# Autodesk Inventor assembly: 0070.011
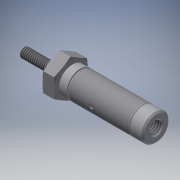
[picture p0: Inventor's stored thumbnail of the model, 180x180]
Saved by Autodesk Inventor 2018 (Build 220112000, 112)
## iProperties
Category: PARTsolutions
Company: BIMBA
Created: 2019-01-16
Part Number: 0070.011
Catalog Web Link: www.cadenas.de
Description: Original Line Standard Air Cylinders-Standard Air Cylinders
Vendor: BIMBA
Document SubType Name: Assembly
Designer: s-4008082
Manufacturer: BIMBA
Mass: 2.26488 g
Surface Area: 33.2461 cm^2
Volume: 2.26488 cm^3
Density: 1 g/cm^3
Title: 0070.011
Author: Cadenas PARTsolutions
Comments: Standard Air Cylinders
PSOL_IDENT_0: {$CADENAS_DATA\23d-libs\bimba\bimba\bimba_imperial\bimba_full_line\original_line_cylinders\standard_
PSOL_IDENT_1: air_cylinders\standard_air_cylinder_asmtab.prj},324 {VTYP=3D},{STYP=ASSTAB},{NB=0070.011},{LINA=0070
PSOL_IDENT_2: .011},{NN=Original Line Standard Air Cylinders},{DATE=21.03.2018 14:31:21},{GEOMDATE=19.03.2018 11:3
PSOL_IDENT_3: 9:15},{VERSION=},{LINEID=20},{WBVAR=STROKE,ACTING,MNT,DER,NR,BM,CO,OO,VO,M,EE,EEL,K,Q,Y,G,T,HL,B,H,S
PSOL_IDENT_4: ER,SR,NT,W,STPT1,STPT2,STPT3,STPT4,MB,PB,PRC,TB,MN},{WBNUMERIC=STROKE,EEL}  {NB=0070.011},{LINA=0070
PSOL_IDENT_5: .011},{KT=DUMMY},{PN=0070.011},{PNC=0070.011},{PNA=(NO ACCESSORIES)},{DASH=},{BORE1=0.31250000},{BOR
PSOL_IDENT_6: E=5/16\" (007)},{BOREPN=007},{STROKE=0.011},{STROKEALG=[0.011:50/0.001]},{STROKE1=0.011},{ACTING=},{
PSOL_IDENT_7: ACTINGALG= '' , 'Single Acting (SA)' , 'R' , 'Reverse Single Acting (SA)' , 'D' , 'Double Acting (SA
PSOL_IDENT_8: )' },{ACTINGPN=},{MNT=},{MNTALG= '' , 'Front Nose Mounting (SA)' , 'XP' , 'Double End or Rear Pivot
PSOL_IDENT_9: Mounting (SA)' },{TYPE=},{MNTPN=},{DER=},{DERALG= '' , 'N/A' },{NR=},{NRALG= '' , 'N/A' },{NRPN=},{B
PSOL_IDENT_10: M=},{BMALG= '' , 'N/A' },{BMPN=},{CO=},{COALG= '' , 'N/A' },{OO=},{OOALG= '', 'N/A' },{OOPN=},{VO=Z}
PSOL_IDENT_11: ,{VOALG= 'Z' , 'N/A' },{VOPN=},{OOVOPN=},{M=},{MALG= '', 'Without Magnet', 'M', 'With Magnet' },{EE=
PSOL_IDENT_12: },{EEL=0.000},{EEMAX=49.9890},{EEALG= '', 'Without Extra Extension', 'EE', 'With Extra Extension' },
PSOL_IDENT_13: {EELALG=0},{EEPN=},{EEPN1=0.000},{K=},{KALG= '' , 'N/A' },{KPN=},{Q=},{QALG= '' , 'Standard Port' , '
PSOL_IDENT_14: Q' , 'Side Port' },{QPN=},{Y=},{YALG= '' , 'N/A' },{YPN=},{YCON=},{F=},{FALG= '', 'Non-Coated (Stand
PSOL_IDENT_15: ard)', 'F', 'Molycoated' },{FPN=},{G=},{GPN=},{GPN99=},{T=},{TALG= '' , 'Standard -20° to 200°F (-29
PSOL_IDENT_16: ° to 95°C)' , 'N' , 'Low Temperature' , 'V' , 'High Temperature' },{NPN=},{VPN=},{HL=},{HLALG= '' , '
PSOL_IDENT_17: N/A' },{B=},{BALG= '' , 'Standard Bumpers' },{BPN=},{H=},{HALG= '', 'N/A' },{HPN=},{SER=},{SERALG= ''
PSOL_IDENT_18: , 'N/A' },{SR=},{SRALG= '' , 'Standard Stainless Steel' },{SRPN=},{SRCON=0},{NT=},{NTPN=},{W=},{WAL
PSOL_IDENT_19: G= '' , 'N/A' },{WPN=},{E=},{EALG= '' , 'Standard Seals/Lube' , 'E' , 'Non-Lube Seals/Lube' },{EPN=}
PSOL_IDENT_20: ,{ST=},{STALG= '' , 'N/A' },{STPT1=},{STPT1ALG= '' , 'N/A' },{STPT2=},{STPT2ALG= '' , 'N/A' },{STPT3=
PSOL_IDENT_21: },{STPT3ALG= '' , 'N/A' },{STPT4=},{STPT4ALG= '' , 'N/A' },{STPN=},{MB=},{MBALG= '' , 'Without Mount
PSOL_IDENT_22: ing Bracket' , 'F,D-26731' , 'D-26731 (front)' },{MBPN=},{MBPNALL=D-26731},{MBPNALLREAR=},{PB=},{PBA
PSOL_IDENT_23: LG= '' , 'N/A' },{PBPN=},{PBPNALL=},{PRC=},{PRCALG= '' , 'W/out Pivot Rod Clevis' , 'F,D-26690' , 'D
PSOL_IDENT_24: -26690 (front)' },{PRCPN=},{PRCPNALL=D-26690},{TB=},{TBALG= '' , 'N/A' },{TBPN=},{TBPNALL=},{MN=},{M
PSOL_IDENT_25: NALG= '' , 'N/A' },{MNPN=},{MNCONF=},{MNCONR=},{TLEN=0.7975},{FRAC=1.3810},{RGCON=},{RGDACCON=},{RHC
PSOL_IDENT_26: ON=},{RHCON1=},{RHCONON=1},{RHACCON=},{FNUTCON=1},{RNUTCON=0},{FNUTPN=D-344},{RNUTPN=},{FNUTTRANS=0.
PSOL_IDENT_27: 0000},{RNUTTRANS=0.0000},{VHOLECON=2},{A1=0.6250},{A1N=0.6250},{A1P=0.8450},{A1B=0.9060},{A4=0.2550}
PSOL_IDENT_28: ,{A4N=0.2550},{A4P=0.1585},{A5=0.0220},{A1H=0.328},{A1NH=0.3280},{A1PH=0.8750},{A1BH=0.0000},{A1SH=0
PSOL_IDENT_29: .0000},{A2H=0.1585},{A2NH=0.1585},{LENGTH=1.1200},{LENGTH1=1.1200},{LENGTH2=1.6500},{MUL=0.0083},{MU
PSOL_IDENT_30: L11=0.0083},{MUL22=0.01375},{MUL33=0.0083},{MUL2=0.7500},{MUL211=0.7500},{MUL222=1.2500},{MUL233=0.7
PSOL_IDENT_31: 500},{SSS=0.0110},{RGLEN=0.3920},{RHLEN=0.1915},{SSS1=1.0000},{A13=0.7190},{DIF=0.0000},{G5=0.0000},
PSOL_IDENT_32: {ON=0},{SSADD=0.0000},{BADD=0.0000},{MADD=0.0000},{NVADD=0.0000},{TRACKL=0.4915},{TRACKCON=D-74168},
PSOL_IDENT_33: {TRIMCON=0},{TRIMCON1=0},{PINCON=},{FSPACE=0.2998},{SPACE=0.0179},{TEXT=0.0313},{S1=0.5000},{D1=0.35
PSOL_IDENT_34: 90},{D1N=0.3590},{D1B=0.6050},{D1P=0.0000},{FA=0.440},{RA=0.0000},{PPATH=standard_air_cylinder_asmtp
PSOL_IDENT_35: l.prj},{MATALGHTML=<b>Standard Original Line:</b><dl><dt>Rod:</dt><dd>- Stainless Steel</dd><dd>&nbs
PSOL_IDENT_36: p;&nbsp;(5/16 9/16 Bores)</dd><dd>- High Strength Carbon Steel</dd><dd>&nbsp;&nbsp;(3/4 3 Bore)</dd>
PSOL_IDENT_37: <dd>- Stainless Steel</dd><dd>&nbsp;&nbsp;(X style DXP/DX/DXDE)</dd><dt>Bearings:</dt><dd>- Sintered
PSOL_IDENT_38: Bronze</dd><dt>Body:</dt><dd>- 304 Stainless Steel</dd><dt>End Caps:</dt><dd>- Aluminum</dd><dt>Sea
PSOL_IDENT_39: ls:</dt><dd>- Buna N</dd></dl>},{ASSCFGPRA=007},{MBPNA=},{MNPNA=},{PRCPNA=},{ASSOPTACC=STPT4},{A=1.3
PSOL_IDENT_40: 8},{HADD=0.0000},{WFL=0},{QADD=0.000},{QADD1=0.200},{TEST=0.0000},{MNTB=},{STDNUTF=1},{STDNUTR=0},{S
PSOL_IDENT_41: TRK2D=0},{X2D=2},{STROKESW=0.011},{EESW=0.000},{FCD=0},{BCD=0},{RCD=0},{CUSTADD=0.000},{FT=#5-40},{F
PSOL_IDENT_42: T1=#5-40},{FT2=3/8-24 UNF-2A},{PORT=#10-32},{FT11=1/2-28 UNF-2A},{FT12=3/8-24 UNF-2A},{B1=}
NN: Original Line Standard Air Cylinders
NT: Standard Male Thread
NB: 0070.011
NBSYN: $PNC.
LINA: 0070.011
PN: 0070.011
PNA: (NO ACCESSORIES)
BORE: 5/16" (007)
STROKE: 0.011
ACTING: Standard Single
MNT: Standard Front Nose
DER: N/A
NR: N/A
BM: N/A
CO: N/A
OO: N/A
VO: N/A
M: Without Magnet Piston
EE: Standard Rod Extension
EEL: 0
K: N/A
Q: Standard Axial Port
Y: N/A
G: Standard Grease Lube
T: Standard -20° to 200°F (-29° to 95°C)
HL: N/A
B: Standard Bumpers
H: N/A
SER: N/A
SR: Standard Stainless Steel
W: N/A
STPT1: N/A
STPT2: N/A
STPT3: N/A
STPT4: N/A
MB: Without Mounting Bracket
PB: N/A
PRC: Without Piston Rod Clevis
TB: N/A
MN: N/A
A: 1.38
SUPPLIER: BIMBA
ARTICLENO: 0070.011
BOMINFO: 0070.011
CREATOR: CADENAS GmbH
## Documents named in this file (7)
- C:\Users\s-4008082\Downloads\hatch\0070_011.iam
- C:\Users\s-4008082\Downloads\hatch\0070_0110000000_0_dummy.ipt
- C:\Users\s-4008082\Downloads\hatch\007000-0_rod_guide.ipt
- C:\Users\s-4008082\Downloads\hatch\007-0_79752.ipt
- C:\Users\s-4008082\Downloads\hatch\0070000_rear_head.ipt
- C:\Users\s-4008082\Downloads\hatch\D-344.ipt
- C:\Users\s-4008082\Downloads\hatch\0070_0110000_rod.ipt
## Components (6 placed, 6 different names)
1. 0070_0110000000_0_dummy:1 — dummy_XY@1 <-> rod_guide_XY@2, dummy_Z@1 <-> rod_guide_Z@2, dummy_YZ@1 <-> rod_guide_YZ@2
2. 007000-0_rod_guide:1 — dummy_XY@1 <-> rod_guide_XY@2, dummy_Z@1 <-> rod_guide_Z@2, dummy_YZ@1 <-> rod_guide_YZ@2, to_tube_XY@2 <-> tube_front_XY@3, to_tube_Z@2 <-> tube_front_Z@3, to_tube_YZ@2 <-> tube_front_YZ@3, to_nut_XY@2 <-> NUT_XY@5, to_nut_Z@2 <-> NUT_Z@5, to_nut_YZ@2 <-> NUT_YZ@5, to_rod_XY@2 <-> rod_cp_XY@6, to_rod_Z@2 <-> rod_cp_Z@6
3. 007-0_79752:1 — to_tube_XY@2 <-> tube_front_XY@3, to_tube_Z@2 <-> tube_front_Z@3, to_tube_YZ@2 <-> tube_front_YZ@3, tube_rear_XY@3 <-> to_tube_XY@4, tube_rear_Z@3 <-> to_tube_Z@4, tube_rear_YZ@3 <-> to_tube_YZ@4
4. 0070000_rear_head:1 — tube_rear_XY@3 <-> to_tube_XY@4, tube_rear_Z@3 <-> to_tube_Z@4, tube_rear_YZ@3 <-> to_tube_YZ@4
5. D-344:1 — to_nut_XY@2 <-> NUT_XY@5, to_nut_Z@2 <-> NUT_Z@5, to_nut_YZ@2 <-> NUT_YZ@5
6. 0070_0110000_rod:1 — to_rod_XY@2 <-> rod_cp_XY@6, to_rod_Z@2 <-> rod_cp_Z@6
## Relationships (14: Flush 5, Mate 5, Angle 4)
- dummy_XY@1 <-> rod_guide_XY@2 [Flush]: 0070_0110000000_0_dummy:1 ↔ 007000-0_rod_guide:1
- dummy_Z@1 <-> rod_guide_Z@2 [Mate]: 0070_0110000000_0_dummy:1 ↔ 007000-0_rod_guide:1
- dummy_YZ@1 <-> rod_guide_YZ@2 [Angle] (0 deg): 0070_0110000000_0_dummy:1 ↔ 007000-0_rod_guide:1
- to_tube_XY@2 <-> tube_front_XY@3 [Flush]: 007000-0_rod_guide:1 ↔ 007-0_79752:1
- to_tube_Z@2 <-> tube_front_Z@3 [Mate]: 007000-0_rod_guide:1 ↔ 007-0_79752:1
- to_tube_YZ@2 <-> tube_front_YZ@3 [Angle] (0 deg): 007000-0_rod_guide:1 ↔ 007-0_79752:1
- tube_rear_XY@3 <-> to_tube_XY@4 [Flush]: 007-0_79752:1 ↔ 0070000_rear_head:1
- tube_rear_Z@3 <-> to_tube_Z@4 [Mate]: 007-0_79752:1 ↔ 0070000_rear_head:1
- tube_rear_YZ@3 <-> to_tube_YZ@4 [Angle] (0 deg): 007-0_79752:1 ↔ 0070000_rear_head:1
- to_nut_XY@2 <-> NUT_XY@5 [Flush]: 007000-0_rod_guide:1 ↔ D-344:1
- to_nut_Z@2 <-> NUT_Z@5 [Mate]: 007000-0_rod_guide:1 ↔ D-344:1
- to_nut_YZ@2 <-> NUT_YZ@5 [Angle] (0 deg): 007000-0_rod_guide:1 ↔ D-344:1
- to_rod_XY@2 <-> rod_cp_XY@6 [Flush]: 007000-0_rod_guide:1 ↔ 0070_0110000_rod:1
- to_rod_Z@2 <-> rod_cp_Z@6 [Mate]: 007000-0_rod_guide:1 ↔ 0070_0110000_rod:1
